# Autodesk Inventor assembly: ConveyorCrossFrame_20Jan
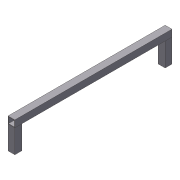
[picture p0: Inventor's stored thumbnail of the model, 180x180]
Saved by Autodesk Inventor 2012 (Build 160160000, 160)
## iProperties
Created: 2012-01-20
Part Number: ConveyorCrossFrame_20Jan
Document SubType Name: Assembly
Designer: JesseK
Mass: 310.585 g
Surface Area: 1452.94 cm^2
Volume: 114.607 cm^3
Density: 2.71 g/cm^3
Author: JesseK
## Documents named in this file (3)
- Z:\UserData\Documents\Inventor\team1885frc\Robot2012\Drawings\ConveyorCrossFrame_20Jan.iam
- Z:\UserData\Documents\Inventor\team1885frc\Robot2012\DriveTrain\Frame_FrontCrossRail.ipt
- Z:\UserData\Documents\Inventor\team1885frc\Robot2012\DriveTrain\Frame_FrontVerticalSupport_forFrontCrossbar.ipt
## Components (3 placed, 2 different names)
1. Frame_FrontCrossRail:1 — Mate:1, Flush:1, Mate:2, Mate:3, Flush:2, Mate:4
2. Frame_FrontVerticalSupport_forFrontCrossbar:1 — Mate:3, Flush:2, Mate:4
3. Frame_FrontVerticalSupport_forFrontCrossbar:2 — Mate:1, Flush:1, Mate:2
## Relationships (6: Mate 4, Flush 2)
- Mate:1: Frame_FrontCrossRail:1 ↔ Frame_FrontVerticalSupport_forFrontCrossbar:2
- Flush:1: Frame_FrontCrossRail:1 ↔ Frame_FrontVerticalSupport_forFrontCrossbar:2
- Mate:2: Frame_FrontCrossRail:1 ↔ Frame_FrontVerticalSupport_forFrontCrossbar:2
- Mate:3: Frame_FrontCrossRail:1 ↔ Frame_FrontVerticalSupport_forFrontCrossbar:1
- Flush:2: Frame_FrontCrossRail:1 ↔ Frame_FrontVerticalSupport_forFrontCrossbar:1
- Mate:4: Frame_FrontCrossRail:1 ↔ Frame_FrontVerticalSupport_forFrontCrossbar:1
